# Autodesk Inventor assembly: Rear_Frame_Fixer
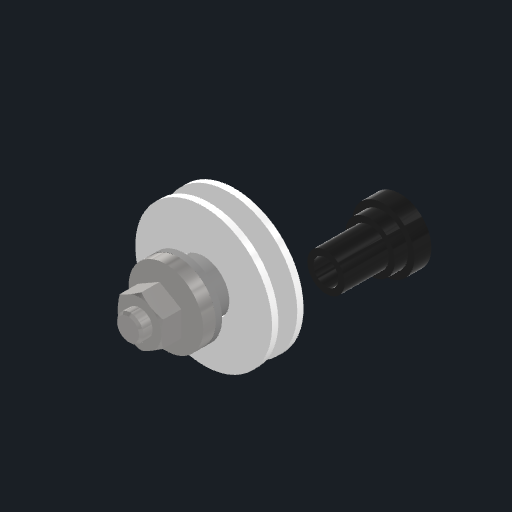
[picture p0: Inventor's stored thumbnail of the model, 512x512]
Saved by Autodesk Inventor 2024.3 (Build 283343000, 343)
## iProperties
Created: 2024-01-28
Part Number: Rear_Frame_Fixer
Document SubType Name: Assembly
Designer: 김대겸
Author: 김대겸
## Documents named in this file (7)
- C:\Users\ASUS\Desktop\Anti_Backlash_Structure_OP\v2_Frame\Rear_Frame_Fixer.iam
- C:\Users\ASUS\Desktop\ABD_2024_Eindhoven\MISUMI\C-WSSA12-4-2.ipt
- C:\Users\ASUS\Desktop\ABD_2024_Eindhoven\MISUMI\TT-0822-10.ipt
- C:\Users\ASUS\Desktop\ABD_2024_Eindhoven\MISUMI\80F-0606.ipt
- C:\Users\ASUS\Desktop\ABD_2024_Eindhoven\MISUMI\CSHCS-SUSTBS-M4-20_214.ipt
- C:\Users\ASUS\Desktop\Anti_Backlash_Structure_OP\v2_Frame\Handmade tiered cover_9mm.ipt
- C:\Users\ASUS\Desktop\ABD_2024_Eindhoven\MISUMI\SLBNR4.ipt
## Components (8 placed, 6 different names)
1. C-WSSA12-4-2:1
2. TT-0822-10:1
3. 80F-0606:1
4. TT-0822-10:2
5. CSHCS-SUSTBS-M4-20_214:1 — 메이트:5
6. Handmade tiered cover_9mm:1
7. SLBNR4:1 — 메이트:5
8. Handmade tiered cover_9mm:2
## Relationships (5: Mate 4, Insert 1)
- [Insert]: C-WSSA12-4-2:1 ↔ 80F-0606:1
- [Mate]: CSHCS-SUSTBS-M4-20_214:1 ↔ Handmade tiered cover_9mm:1
- [Mate]: TT-0822-10:2 ↔ Handmade tiered cover_9mm:1
- [Mate]: TT-0822-10:2 ↔ Handmade tiered cover_9mm:1
- 메이트:5 [Mate]: CSHCS-SUSTBS-M4-20_214:1 ↔ SLBNR4:1
## Named parameters: d710_d709 = 0 mm
